# Autodesk Inventor assembly: reza2
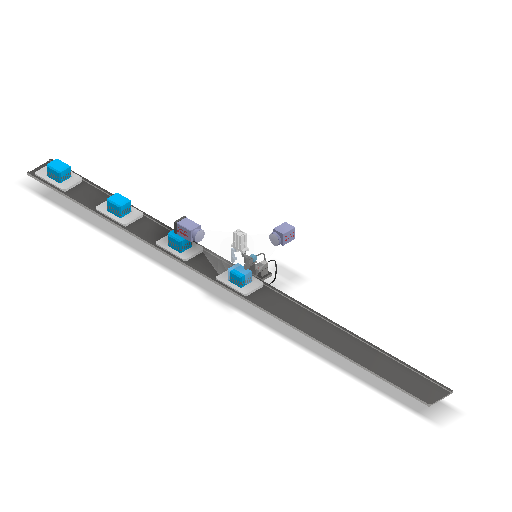
[picture p0: Inventor's stored thumbnail of the model, 512x512]
Saved by Autodesk Inventor 2025 (Build 290162000, 162)
## iProperties
Created: 2024-09-26
Part Number: reza2
Document SubType Name: Assembly
Designer: DMIADX
Author: DMIADX
## Documents named in this file (15)
- C:\Users\DMIADX\Documents\chuck\reza2.iam
- C:\Users\DMIADX\Documents\chuck\chuck.ipt
- C:\Users\DMIADX\Documents\chuck\chuck_MIR.ipt
- C:\Users\DMIADX\Documents\chuck\MHZL2-20D\MHZL2-20D.ipt
- C:\Users\DMIADX\Documents\chuck\Connector2.ipt
- C:\Users\DMIADX\Documents\Inventor\Content Center Files\R2025\en-US\ISO 4762(2)\ISO 4762 - M3 x 12ISO.ipt
- C:\Users\DMIADX\Documents\chuck\pallet.ipt
- C:\Users\DMIADX\Documents\chuck\part.ipt
- C:\Users\DMIADX\Documents\chuck\CAMERA TERMINAL.ipt
- C:\Users\DMIADX\Documents\chuck\CAMERA.ipt
- C:\Users\DMIADX\Documents\chuck\flash.ipt
- C:\Users\DMIADX\Documents\chuck\jalur.ipt
- C:\Users\DMIADX\Documents\chuck\holder sensor.ipt
- C:\Users\DMIADX\Documents\chuck\cover.ipt
- C:\Users\DMIADX\Documents\chuck\sensor.ipt
## Components (26 placed, 14 different names)
1. chuck:1 — Mate:3, Mate:5, Mate:6, Insert:1, Insert:2
2. chuck_MIR:1 — Mate:7, Mate:8, Mate:9, Insert:3, Insert:4, chuck naik
3. MHZL2-20D:1 — Mate:1, Mate:2, chuck 1 open, chuck 2 open, Flush:4, Flush:6
4. Connector2:1 — Flush:1, Mate:1, Mate:2, Flush:2, Mate:3, chuck 1 open, Mate:5, Mate:6
5. Connector2:2 — Flush:1, Flush:2, chuck 2 open, Mate:7, Mate:8, Mate:9
6. ISO 4762 M3 x 12:1 — Insert:1
7. ISO 4762 M3 x 12:2 — Insert:2
8. ISO 4762 M3 x 12:3 — Insert:4
9. ISO 4762 M3 x 12:4 — Insert:3
10. pallet:1 — Flush:7, geser palet, Mate:10, Mate:29
11. part:1 — part naik, Flush:9, geser part
12. pallet:2 — Mate:12, Flush:12, Flush:14, Mate:24
13. part:2 — Mate:13, Flush:11, Flush:13
14. CAMERA TERMINAL:1 — Flush:16, Mate:16, Flush:17, Insert:6
15. CAMERA:1 — Flush:15, Mate:14, Mate:15, Insert:5
16. flash:1 — Insert:5
17. flash:2 — Insert:6
18. jalur:1 — Mate:17, Mate:18, Flush:18, Mate:19, Mate:23, Mate:28, Mate:30
19. pallet:3 — Mate:19, Mate:20, Mate:21, Mate:22, Mate:23, Mate:24
20. part:3 — Mate:20, Mate:21, Mate:22
21. pallet:4 — Mate:28, Mate:29, Mate:30
22. part:4
23. holder sensor:1 — Mate:31, Mate:32, Flush:19, Mate:33, Flush:20, Flush:21, Mate:34, Flush:22, Flush:23
24. cover:1 — Mate:35, Mate:36, Mate:37
25. sensor:1 — Mate:34, Flush:22, Flush:23
26. sensor:2 — Mate:33, Flush:20, Flush:21, Mate:35, Mate:36, Mate:37
## Relationships (66: Mate 37, Flush 23, Insert 6)
- Flush:1: Connector2:1 ↔ Connector2:2
- Mate:1: MHZL2-20D:1 ↔ Connector2:1
- Mate:2: MHZL2-20D:1 ↔ Connector2:1
- Flush:2: Connector2:1 ↔ Connector2:2
- Mate:3: chuck:1 ↔ Connector2:1
- chuck 1 open [Flush]: MHZL2-20D:1 ↔ Connector2:1
- chuck 2 open [Mate]: MHZL2-20D:1 ↔ Connector2:2
- Mate:5: chuck:1 ↔ Connector2:1
- Mate:6: chuck:1 ↔ Connector2:1
- Mate:7: chuck_MIR:1 ↔ Connector2:2
- Mate:8: chuck_MIR:1 ↔ Connector2:2
- Mate:9: chuck_MIR:1 ↔ Connector2:2
- Insert:1: chuck:1 ↔ ISO 4762 M3 x 12:1
- Insert:2: chuck:1 ↔ ISO 4762 M3 x 12:2
- Insert:3: chuck_MIR:1 ↔ ISO 4762 M3 x 12:4
- Insert:4: chuck_MIR:1 ↔ ISO 4762 M3 x 12:3
- Flush:4: MHZL2-20D:1
- chuck naik [Flush] (80 mm): chuck_MIR:1
- Flush:6: MHZL2-20D:1
- Flush:7: pallet:1
- geser palet [Flush] (300 mm): pallet:1
- Mate:10: pallet:1
- part naik [Mate] (-8 mm): part:1
- Flush:9: part:1
- geser part [Flush] (300 mm): part:1
- Mate:12: pallet:2
- Mate:13 (-8 mm): part:2
- Flush:11: part:2
- Flush:12: pallet:2
- Flush:13 (600 mm): part:2
- Flush:14 (600 mm): pallet:2
- Flush:15: CAMERA:1
- Mate:14 (-100 mm): CAMERA:1
- Mate:15 (250 mm): CAMERA:1
- Flush:16: CAMERA TERMINAL:1
- Mate:16 (-100 mm): CAMERA TERMINAL:1
- Flush:17 (300 mm): CAMERA TERMINAL:1
- Insert:5: CAMERA:1 ↔ flash:1
- Insert:6: CAMERA TERMINAL:1 ↔ flash:2
- Mate:17: jalur:1
- Mate:18: jalur:1
- Flush:18: jalur:1
- Mate:19: jalur:1 ↔ pallet:3
- Mate:20: pallet:3 ↔ part:3
- Mate:21: pallet:3 ↔ part:3
- Mate:22: pallet:3 ↔ part:3
- Mate:23: jalur:1 ↔ pallet:3
- Mate:24 (150 mm): pallet:2 ↔ pallet:3
- [Mate]: pallet:4 ↔ part:4
- [Mate]: pallet:4 ↔ part:4
- [Mate]: pallet:4 ↔ part:4
- Mate:28: jalur:1 ↔ pallet:4
- Mate:29 (150 mm): pallet:1 ↔ pallet:4
- Mate:30: jalur:1 ↔ pallet:4
- Mate:31: holder sensor:1
- Mate:32: holder sensor:1
- Flush:19 (-85 mm): holder sensor:1
- Mate:33: holder sensor:1 ↔ sensor:2
- Flush:20 (2.5 mm): holder sensor:1 ↔ sensor:2
- Flush:21: holder sensor:1 ↔ sensor:2
- Mate:34: holder sensor:1 ↔ sensor:1
- Flush:22: holder sensor:1 ↔ sensor:1
- Flush:23 (2.5 mm): holder sensor:1 ↔ sensor:1
- Mate:35: cover:1 ↔ sensor:2
- Mate:36: cover:1 ↔ sensor:2
- Mate:37: cover:1 ↔ sensor:2
## Named parameters: d61_d56 = 0 mm, d62_d57 = 0 mm, d63_d58 = 0 mm
